# Autodesk Inventor assembly: Payload
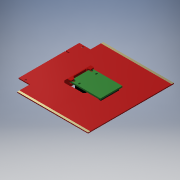
[picture p0: Inventor's stored thumbnail of the model, 180x180]
Saved by Autodesk Inventor 2018 (Build 220112000, 112)
## iProperties
Created: 2018-07-04
Part Number: Payload
Document SubType Name: Assembly
Designer: Bradley
Author: Bradley
## Documents named in this file (7)
- D:\Users\Bradley\Documents\CougsInSpace\CougSat1-Hardware\CougSat1-Payload\CADModel\Native\Payload.iam
- D:\Users\Bradley\Documents\CougsInSpace\CougSat1-Hardware\CougSat1-Payload\CADModel\Native\Payload_PCB.ipt
- D:\Users\Bradley\Documents\CougsInSpace\Resources\ComponentModels\Electronics\Module_ArducamMini-Rev.ipt
- D:\Users\Bradley\Documents\CougsInSpace\Resources\ComponentModels\Hardware\Lens_M12_1.70mm-f2.8.ipt
- D:\Users\Bradley\Documents\CougsInSpace\Resources\ComponentModels\Hardware\LensMount_M12-20mm.ipt
- D:\Users\Bradley\Documents\CougsInSpace\CougSat1-Hardware\CougSat1-Payload\CADModel\Native\Payload_CameraSupport.ipt
- D:\Users\Bradley\Documents\CougsInSpace\Resources\ComponentModels\Fasteners\Bolt_M2x0.4_4mm_SH.ipt
## Components (7 placed, 6 different names)
1. Payload_PCB:1 — Mate:1, Insert:4, Insert:5, Insert:6, Insert:7
2. Module_ArducamMini-Rev:1 — Mate:1, Mate:2, Insert:1, Insert:2, Insert:3, Mate:4
3. Lens_M12_1.70mm-f2.8:1 — Insert:1
4. LensMount_M12-20mm:1 — Insert:2, Insert:3
5. Payload_CameraSupport:1 — Insert:4, Insert:5, Mate:4
6. Bolt_M2x0.4_4mm_SH:1 — Insert:6
7. Bolt_M2x0.4_4mm_SH:2 — Insert:7
## Relationships (10: Insert 7, Mate 3)
- Mate:1: Payload_PCB:1 ↔ Module_ArducamMini-Rev:1
- Mate:2: Module_ArducamMini-Rev:1
- Insert:1: Module_ArducamMini-Rev:1 ↔ Lens_M12_1.70mm-f2.8:1
- Insert:2: Module_ArducamMini-Rev:1 ↔ LensMount_M12-20mm:1
- Insert:3: Module_ArducamMini-Rev:1 ↔ LensMount_M12-20mm:1
- Insert:4: Payload_PCB:1 ↔ Payload_CameraSupport:1
- Insert:5: Payload_PCB:1 ↔ Payload_CameraSupport:1
- Mate:4: Module_ArducamMini-Rev:1 ↔ Payload_CameraSupport:1
- Insert:6: Payload_PCB:1 ↔ Bolt_M2x0.4_4mm_SH:1
- Insert:7: Payload_PCB:1 ↔ Bolt_M2x0.4_4mm_SH:2
